# Autodesk Inventor assembly: PortaPiezasV2
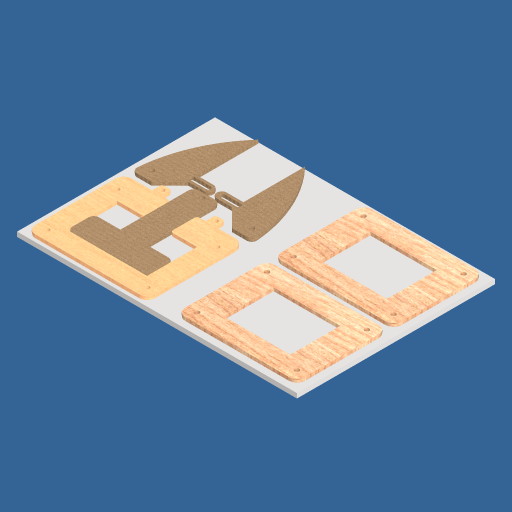
[picture p0: Inventor's stored thumbnail of the model, 512x512]
Saved by Autodesk Inventor 2023.2 (Build 272271000, 271)
## iProperties
Created: 2022-11-22
Part Number: PortaPiezasV2
Document SubType Name: Assembly
Designer: Daniel Peña
Author: Daniel Peña
## Documents named in this file (6)
- E:\Daniel DiscoA\Documents\UNAL\ProyectoRobotica\CAD\V3 - BigChungus\PortaPiezasV2.iam
- E:\Daniel DiscoA\Documents\UNAL\ProyectoRobotica\CAD\Part3.ipt
- E:\Daniel DiscoA\Documents\UNAL\ProyectoRobotica\CAD\V3 - BigChungus\Dedo-BC.ipt
- E:\Daniel DiscoA\Documents\UNAL\ProyectoRobotica\CAD\V3 - BigChungus\MarcoBC.ipt
- E:\Daniel DiscoA\Documents\UNAL\ProyectoRobotica\CAD\V3 - BigChungus\TapaBC.ipt
- E:\Daniel DiscoA\Documents\UNAL\ProyectoRobotica\CAD\V3 - BigChungus\PistonBC.ipt
## Components (7 placed, 5 different names)
1. Part3:1 — Flush:1, Flush:2, Flush:3, Flush:4, Flush:5, Flush:6, Flush:8, Flush:9, Flush:11, Flush:12
2. Dedo-BC:1 — Flush:3, Flush:7, Mate:3, Mate:4
3. Dedo-BC:2 — Flush:2, Flush:7, Mate:3
4. MarcoBC:1 — Flush:4, Mate:1, Mate:2, Flush:8, Flush:9, Mate:4
5. TapaBC:1 — Flush:1, Mate:5, Flush:10, Flush:11, Flush:12
6. TapaBC:2 — Flush:6, Mate:5, Flush:10
7. PistonBC:1 — Flush:5, Mate:1, Mate:2
## Relationships (17: Flush 12, Mate 5)
- Flush:1 (-5 mm): Part3:1 ↔ TapaBC:1
- Flush:2 (-5 mm): Part3:1 ↔ Dedo-BC:2
- Flush:3 (-5 mm): Part3:1 ↔ Dedo-BC:1
- Flush:4 (-5 mm): Part3:1 ↔ MarcoBC:1
- Flush:5 (-5 mm): Part3:1 ↔ PistonBC:1
- Flush:6 (-5 mm): Part3:1 ↔ TapaBC:2
- Mate:1: MarcoBC:1 ↔ PistonBC:1
- Mate:2: MarcoBC:1 ↔ PistonBC:1
- Flush:7: Dedo-BC:1 ↔ Dedo-BC:2
- Mate:3 (70 mm): Dedo-BC:1 ↔ Dedo-BC:2
- Flush:8 (10 mm): Part3:1 ↔ MarcoBC:1
- Flush:9 (-5 mm): Part3:1 ↔ MarcoBC:1
- Mate:4 (38 mm): Dedo-BC:1 ↔ MarcoBC:1
- Mate:5 (10 mm): TapaBC:1 ↔ TapaBC:2
- Flush:10: TapaBC:1 ↔ TapaBC:2
- Flush:11 (10 mm): Part3:1 ↔ TapaBC:1
- Flush:12 (10 mm): Part3:1 ↔ TapaBC:1
